# Autodesk Inventor assembly: paint platform assy2
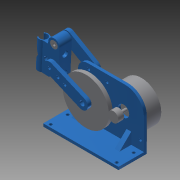
[picture p0: Inventor's stored thumbnail of the model, 180x180]
Saved by Autodesk Inventor 2013 SP2 (Build 170200200, 200)
## iProperties
Created: 2017-01-29
Part Number: paint platform assy2
Document SubType Name: Assembly
Designer: Herman de Vries
Author: Herman de Vries
## Documents named in this file (9)
- E:\_hdv\Projects\PainterBot\paint platform assy2.iam
- E:\_hdv\Projects\PainterBot\paint holder 2.ipt
- E:\_hdv\Projects\PainterBot\stepper motor 1.ipt
- E:\_hdv\Projects\PainterBot\gear.ipt
- E:\_hdv\Projects\PainterBot\z axis arm1.ipt
- E:\_hdv\Projects\PainterBot\z axis arm3.ipt
- E:\_hdv\Projects\PainterBot\z axis arm2.ipt
- E:\_hdv\Projects\PainterBot\bearing 3mmx8mmx5mm.ipt
- E:\_hdv\Projects\PainterBot\brush clip.ipt
## Components (11 placed, 8 different names)
1. paint holder 2:1 — Insert:1, Insert:8, Insert:9, Insert:10
2. stepper motor 1:1 — Insert:1, Insert:10
3. gear:1 — Insert:4, Insert:5, Insert:9
4. z axis arm1:1 — Insert:8, Mate:1
5. z axis arm3:1 — Mate:1, Insert:11, Insert:12, Insert:13, Insert:14, Insert:15, Insert:16, Insert:17
6. z axis arm2:1 — Insert:4, Insert:5, Insert:11
7. bearing 3mmx8mmx5mm:1 — Insert:12
8. bearing 3mmx8mmx5mm:2 — Insert:13
9. bearing 3mmx8mmx5mm:3 — Insert:14
10. bearing 3mmx8mmx5mm:4 — Insert:15
11. brush clip:1 — Insert:16, Insert:17
## Relationships (14: Insert 13, Mate 1)
- Insert:1: paint holder 2:1 ↔ stepper motor 1:1
- Insert:4: gear:1 ↔ z axis arm2:1
- Insert:5: gear:1 ↔ z axis arm2:1
- Insert:8: paint holder 2:1 ↔ z axis arm1:1
- Insert:9: paint holder 2:1 ↔ gear:1
- Insert:10: paint holder 2:1 ↔ stepper motor 1:1
- Mate:1: z axis arm1:1 ↔ z axis arm3:1
- Insert:11: z axis arm3:1 ↔ z axis arm2:1
- Insert:12: z axis arm3:1 ↔ bearing 3mmx8mmx5mm:1
- Insert:13: z axis arm3:1 ↔ bearing 3mmx8mmx5mm:2
- Insert:14: z axis arm3:1 ↔ bearing 3mmx8mmx5mm:3
- Insert:15: z axis arm3:1 ↔ bearing 3mmx8mmx5mm:4
- Insert:16: z axis arm3:1 ↔ brush clip:1
- Insert:17: z axis arm3:1 ↔ brush clip:1
